# Autodesk Inventor assembly: Wrist
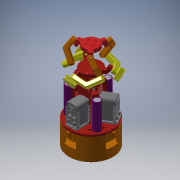
[picture p0: Inventor's stored thumbnail of the model, 180x180]
Saved by Autodesk Inventor 2019 (Build 230136000, 136)
## iProperties
Created: 2022-08-01
Part Number: Wrist
Document SubType Name: Assembly
Designer: zreik
Author: zreik
## Documents named in this file (3)
- D:\Documents\HIAST\4th year\4th Year Project\Design\Current\Wrist.iam
- D:\Documents\HIAST\4th year\4th Year Project\Design\Current\SPM.iam
- D:\Documents\HIAST\4th year\4th Year Project\Design\Current\Base.ipt
## Components (2 placed, 2 different names)
1. SPM:1 [sub-assembly] — Mate:1, Mate:2, Mate:3
2. Base:1 — Mate:1, Mate:2, Mate:3, Mate:4, Flush:1, Mate:5
## Relationships (6: Mate 5, Flush 1)
- Mate:1: SPM:1 ↔ Base:1
- Mate:2: SPM:1 ↔ Base:1
- Mate:3: SPM:1 ↔ Base:1
- Mate:4: Base:1
- Flush:1: Base:1
- Mate:5: Base:1
